# Autodesk Inventor assembly: nc_nhk27
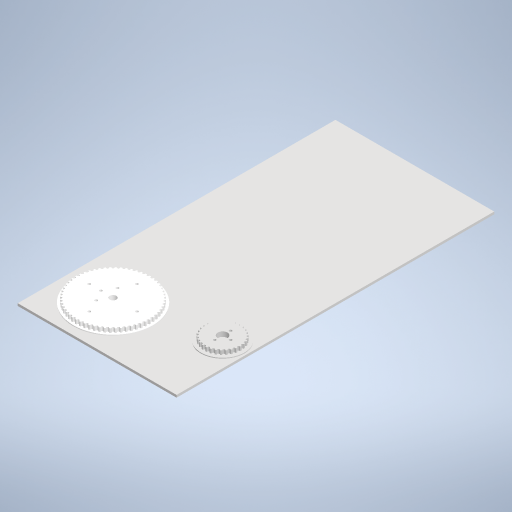
[picture p0: Inventor's stored thumbnail of the model, 512x512]
Saved by Autodesk Inventor 2023 (Build 270158000, 158)
## iProperties
Created: 2022-05-10
Part Number: nc_nhk27
Document SubType Name: Assembly
Designer: yuta
Author: yuta
## Documents named in this file (4)
- C:\Users\yuta\Documents\NHK\nc_nhk27.iam
- C:\Users\yuta\Documents\NHK\NC.port.ipt
- C:\Users\yuta\Documents\NHK\射出_プーリ30.ipt
- C:\Users\yuta\Documents\NHK\射出_プーリ_歯数60.ipt
## Components (3 placed, 3 different names)
1. NC.port:1 — メイト:1, メイト:2, メイト:3, メイト:4, メイト:5
2. 射出_プーリ30:1 — メイト:4, メイト:5
3. 射出_プーリ_歯数60:1 — メイト:1, メイト:2, メイト:3
## Relationships (5: Mate 5)
- メイト:1 [Mate]: NC.port:1 ↔ 射出_プーリ_歯数60:1
- メイト:2 [Mate] (-60 mm): NC.port:1 ↔ 射出_プーリ_歯数60:1
- メイト:3 [Mate] (-60 mm): NC.port:1 ↔ 射出_プーリ_歯数60:1
- メイト:4 [Mate] (-30 mm): NC.port:1 ↔ 射出_プーリ30:1
- メイト:5 [Mate]: NC.port:1 ↔ 射出_プーリ30:1
